# Autodesk Inventor assembly: Stopa v4
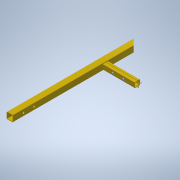
[picture p0: Inventor's stored thumbnail of the model, 180x180]
Saved by Autodesk Inventor 2021 (Build 250183000, 183)
## iProperties
Created: 2024-04-18
Part Number: Stopa v4
Document SubType Name: Assembly
Designer: Michal
Author: Michal
## Documents named in this file (4)
- C:\Users\Michal\Documents\GitHub\PNW_PhotoBoothFrame_3D\Stopa v4.iam
- C:\Users\Michal\Documents\GitHub\PNW_PhotoBoothFrame_3D\Stopa v2 profil 1.ipt
- C:\Users\Michal\Documents\GitHub\PNW_PhotoBoothFrame_3D\M8x15.ipt
- C:\Users\Michal\Documents\GitHub\PNW_PhotoBoothFrame_3D\Stopa v4 profil 1.ipt
## Components (4 placed, 3 different names)
1. Stopa v4 profil 1:1 — Mate:11, Mate:12, Mate:14, Mate:15
2. Stopa v2 profil 1:1 — Mate:12, Mate:13, Flush:5, Mate:15, Mate:16, Mate:17, Mate:18
3. M8x15:1 — Mate:16, Flush:6
4. M8x15:2 — Mate:17, Flush:6, Mate:18
## Relationships (10: Mate 8, Flush 2)
- Mate:11: Stopa v4 profil 1:1
- Mate:12: Stopa v4 profil 1:1 ↔ Stopa v2 profil 1:1
- Mate:13: Stopa v2 profil 1:1
- Flush:5: Stopa v2 profil 1:1
- Mate:14: Stopa v4 profil 1:1
- Mate:15 (150 mm): Stopa v4 profil 1:1 ↔ Stopa v2 profil 1:1
- Mate:16: Stopa v2 profil 1:1 ↔ M8x15:1
- Mate:17: Stopa v2 profil 1:1 ↔ M8x15:2
- Flush:6: M8x15:1 ↔ M8x15:2
- Mate:18 (3 mm): Stopa v2 profil 1:1 ↔ M8x15:2
